# Autodesk Inventor assembly: SSE2B6L-70
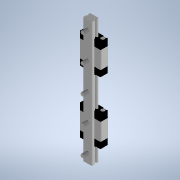
[picture p0: Inventor's stored thumbnail of the model, 180x180]
Saved by Autodesk Inventor 2021 (Build 250183000, 183)
## iProperties
Category: PARTsolutions
Company: MISUMI
Created: 2025-06-07
Part Number: SSE2B6L-70
Catalog Web Link: www.cadenas.de
Description: SSEB, SSEB-MX, SSE2B, SSE2B-MX, RSEB, RSE2B-Miniature Linear Guides Standard Blocks/Light Preload High Grade-L Selectable Type
Vendor: MISUMI
Document SubType Name: Assembly
Designer: psAdmin
Manufacturer: MISUMI
Mass: 2.66105 g
Surface Area: 35.1391 cm^2
Volume: 2.66105 cm^3
Density: 1 g/cm^3
Title: SSE2B6L-70
Author: Cadenas PARTsolutions
Comments: Miniature Linear Guides Standard Blocks/Light Preload High Grade-L Selectable Type
PSOL_IDENT_0: {$CADENAS_DATA/23d-libs/misumi/metric/06_linear_guides/re2b_asmtab.prj},256 {VTYP=3D},{STYP=ASSTAB},
PSOL_IDENT_1: {NB=SSE2B6L-70},{LINA=SSE2B6L-70},{NN=SSEB, SSEB-MX, SSE2B, SSE2B-MX, RSEB, RSE2B},{DATE=04.04.2024
PSOL_IDENT_2: 07:12:35},{GEOMDATE=07.03.2024 00:33:43},{VERSION=},{LINEID=60},{WBVAR=ST,MAT,MX,NOB,GREASE,LS,ALT1,
PSOL_IDENT_3: ALT2,ALT3,ALT4},{WBNUMERIC=LS}  {NB=SSE2B6L-70},{LINA=SSE2B6L-70},{KT=DUMMY},{PN=SSE2B6L-70},{RT=B},
PSOL_IDENT_4: {TYPE=SSE2B},{ST=S},{MAT=S},{MX=},{MXALG= '','w/o MX(Lubrication unit)' },{NOB=2},{H=6},{GREASE=L},{
PSOL_IDENT_5: GREASEALG='','Normal', 'L'  , 'L Type Greased ', 'G', 'G Type Greased', 'Y', 'Y Type Greased', 'H', '
PSOL_IDENT_6: H Type Greased'},{LT=Selectable},{LS=70},{HARD=56HRC~},{W=12},{L1=17.4},{B=8},{C=0},{SLL=M2x1.5},{L2=
PSOL_IDENT_7: 9.7},{K=4.5},{CBB=0.3},{W1=5},{W2=3.5},{H1=4.0},{CAA=0.3},{DD1DD2HH=2.4x3.5x1},{F=15},{G=5.0},{ALT1=
PSOL_IDENT_8: },{ALT1ALG= '', 'w/o MC (Tapped Holes)', '-MC', 'with MC (Tapped Holes)' },{MC=M2.6},{ALT2=},{ALT2L=
PSOL_IDENT_9: 0.0},{ALT2N=0},{M=5},{LL=},{L0=70,85,100,115,130,145},{REC1=   '','Not applicable'    },{ST1='S', 'w
PSOL_IDENT_10: /o Surface Treatment'},{MAT2='S','Stainless Steel'},{ALT3=},{ALT3ALG= '' , 'w/o WC (Pair of Rails)'
PSOL_IDENT_11: , '-WC' , 'with WC (Set Pair of Rails)' },{ALT4=},{ALT4ALG= '','N/A' },{PPATH=seb_series/seb_asmtpl.
PSOL_IDENT_12: prj}
NB: SSE2B6L-70
NN: SSEB, SSEB-MX, SSE2B, SSE2B-MX, RSEB, RSE2B
NT: Miniature Linear Guides Standard Blocks/Light Preload High Grade-L Selectable Type
NBSYN: $PN.
LINA: SSE2B6L-70
CATALOG: Misumi
PN: SSE2B6L-70
ST: w/o Surface Treatment
MAT: Stainless Steel
MX: w/o MX(Lubrication unit)
NOB: 2
H: 6
GREASE: L Type Greased
LS: 70
W: 12
L1: 17.4
B: 8
C: 0
SLL: M2x1.5
L2: 9.7
K: 4.5
CBB: 0.3
W1: 5
W2: 3.5
H1: 4
CAA: 0.3
DD1DD2HH: 2.4x3.5x1
F: 15
G: 5
ALT1: w/o MC (Tapped Holes)
ALT2: Not applicable
ALT3: w/o WC (Pair of Rails)
ALT4: N/A
SUPPLIER: MISUMI
ARTICLENO: SSE2B6L-70
BOMINFO: SSE2B6L-70
CREATOR: CADENAS GmbH
## Documents named in this file (4)
- e:\temp\worker_COMMON_271\temp\tmp_2088_0_gqSUJ\format_0\SSE2B6L-70.iam
- e:\temp\worker_COMMON_271\temp\tmp_2088_0_gqSUJ\format_0\SSE2B6-70_r.ipt
- e:\temp\worker_COMMON_271\temp\tmp_2088_0_gqSUJ\format_0\SSEB6_b.ipt
- e:\temp\worker_COMMON_271\temp\tmp_2088_0_gqSUJ\format_0\M2x6_b.ipt
## Components (8 placed, 3 different names)
1. SSE2B6-70_r:1 — to_block_Z@1 <-> to_rail_Z@2, to_block_YZ@1 <-> to_rail_YZ@2, to_block_2_Z@1 <-> to_rail_Z@3, to_block_2_YZ@1 <-> to_rail_YZ@3, screw_1_Z@1 <-> screw_to_rail_Z@4, screw_1_YZ@1 <-> screw_to_rail_YZ@4, screw_2_Z@1 <-> screw_to_rail_Z@5, screw_2_YZ@1 <-> screw_to_rail_YZ@5, screw_3_Z@1 <-> screw_to_rail_Z@6, screw_3_YZ@1 <-> screw_to_rail_YZ@6, screw_4_Z@1 <-> screw_to_rail_Z@7, screw_4_YZ@1 <-> screw_to_rail_YZ@7, screw_5_Z@1 <-> screw_to_rail_Z@8, screw_5_YZ@1 <-> screw_to_rail_YZ@8
2. SSEB6_b:1 — to_block_Z@1 <-> to_rail_Z@2, to_block_YZ@1 <-> to_rail_YZ@2
3. SSEB6_b:2 — to_block_2_Z@1 <-> to_rail_Z@3, to_block_2_YZ@1 <-> to_rail_YZ@3
4. M2x6_b:1 — screw_1_Z@1 <-> screw_to_rail_Z@4, screw_1_YZ@1 <-> screw_to_rail_YZ@4
5. M2x6_b:2 — screw_2_Z@1 <-> screw_to_rail_Z@5, screw_2_YZ@1 <-> screw_to_rail_YZ@5
6. M2x6_b:3 — screw_3_Z@1 <-> screw_to_rail_Z@6, screw_3_YZ@1 <-> screw_to_rail_YZ@6
7. M2x6_b:4 — screw_4_Z@1 <-> screw_to_rail_Z@7, screw_4_YZ@1 <-> screw_to_rail_YZ@7
8. M2x6_b:5 — screw_5_Z@1 <-> screw_to_rail_Z@8, screw_5_YZ@1 <-> screw_to_rail_YZ@8
## Relationships (14: Mate 7, Angle 7)
- to_block_Z@1 <-> to_rail_Z@2 [Mate]: SSE2B6-70_r:1 ↔ SSEB6_b:1
- to_block_YZ@1 <-> to_rail_YZ@2 [Angle] (0 deg): SSE2B6-70_r:1 ↔ SSEB6_b:1
- to_block_2_Z@1 <-> to_rail_Z@3 [Mate]: SSE2B6-70_r:1 ↔ SSEB6_b:2
- to_block_2_YZ@1 <-> to_rail_YZ@3 [Angle] (0 deg): SSE2B6-70_r:1 ↔ SSEB6_b:2
- screw_1_Z@1 <-> screw_to_rail_Z@4 [Mate]: SSE2B6-70_r:1 ↔ M2x6_b:1
- screw_1_YZ@1 <-> screw_to_rail_YZ@4 [Angle] (0 deg): SSE2B6-70_r:1 ↔ M2x6_b:1
- screw_2_Z@1 <-> screw_to_rail_Z@5 [Mate]: SSE2B6-70_r:1 ↔ M2x6_b:2
- screw_2_YZ@1 <-> screw_to_rail_YZ@5 [Angle] (0 deg): SSE2B6-70_r:1 ↔ M2x6_b:2
- screw_3_Z@1 <-> screw_to_rail_Z@6 [Mate]: SSE2B6-70_r:1 ↔ M2x6_b:3
- screw_3_YZ@1 <-> screw_to_rail_YZ@6 [Angle] (0 deg): SSE2B6-70_r:1 ↔ M2x6_b:3
- screw_4_Z@1 <-> screw_to_rail_Z@7 [Mate]: SSE2B6-70_r:1 ↔ M2x6_b:4
- screw_4_YZ@1 <-> screw_to_rail_YZ@7 [Angle] (0 deg): SSE2B6-70_r:1 ↔ M2x6_b:4
- screw_5_Z@1 <-> screw_to_rail_Z@8 [Mate]: SSE2B6-70_r:1 ↔ M2x6_b:5
- screw_5_YZ@1 <-> screw_to_rail_YZ@8 [Angle] (0 deg): SSE2B6-70_r:1 ↔ M2x6_b:5
